# Autodesk Inventor assembly: sweeper
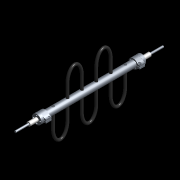
[picture p0: Inventor's stored thumbnail of the model, 180x180]
Saved by Autodesk Inventor 2015 SP1 (Build 190203100, 203)
## iProperties
Created: 2015-01-25
Part Number: sweeper
Document SubType Name: Assembly
Designer: rihoobler
Author: rihoobler
## Documents named in this file (7)
- C:\Users\datenney\Documents\GitHub\CAD\SerenityMk.2\sweeper.iam
- C:\Users\datenney\Documents\GitHub\CAD\SerenityMk.2\Sweeper tube.ipt
- C:\Users\datenney\Documents\GitHub\CAD\SerenityMk.2\Surgical.ipt
- C:\Users\datenney\Documents\GitHub\CAD\SerenityMk.2\Imported Components\tetrix_739077_2012\tetrix_739077_2012.ipt
- C:\Users\datenney\Documents\GitHub\CAD\SerenityMk.2\Imported Components\tetrix_739172_2012\tetrix_739172_2012.iam
- C:\Users\datenney\Documents\GitHub\CAD\SerenityMk.2\Imported Components\tetrix_739088_2012\tetrix_739088_2012.ipt
- C:\Users\datenney\Documents\GitHub\CAD\SerenityMk.2\Imported Components\tetrix_739101_2012\tetrix_739101_2012.ipt
## Components (16 placed, 6 different names)
1. Sweeper tube:1 — Mate:1, Mate:2, Mate:4, Mate:5, Mate:7, Mate:8, Mate:11, Mate:13, Mate:14, Insert:1, Insert:2
2. Surgical:1 — Mate:3, Mate:4, Mate:5, Mate:6
3. Surgical:2 — Mate:6, Mate:7, Mate:8, Mate:9, Mate:10
4. Surgical:3 — Mate:1, Mate:2, Flush:1, Mate:3, Flush:2
5. Surgical:4 — Mate:9, Mate:10, Mate:11, Mate:12
6. Surgical:5 — Mate:12, Mate:13, Mate:14
7. tetrix_739077_2012:1 — Insert:2, Insert:4
8. tetrix_739077_2012:2 — Insert:1, Flush:2, Insert:3
9. tetrix_739172_2012:1 [sub-assembly] — Insert:4, Mate:15, Flush:3, Insert:7
10. tetrix_739172_2012:2 [sub-assembly] — Insert:3, Mate:16, Flush:4, Insert:5
11. tetrix_739088_2012:1 — Mate:16, Flush:4
12. tetrix_739088_2012:2 — Mate:15, Flush:3
13. tetrix_739101_2012:1 — Insert:6
14. tetrix_739101_2012:2 — Insert:5, Insert:6
15. tetrix_739101_2012:3 — Insert:8
16. tetrix_739101_2012:4 — Insert:7, Insert:8
## Relationships (28: Mate 16, Insert 8, Flush 4)
- Mate:1: Sweeper tube:1 ↔ Surgical:3
- Mate:2: Sweeper tube:1 ↔ Surgical:3
- Flush:1: Surgical:3
- Mate:3: Surgical:1 ↔ Surgical:3
- Mate:4: Sweeper tube:1 ↔ Surgical:1
- Mate:5: Sweeper tube:1 ↔ Surgical:1
- Mate:6: Surgical:1 ↔ Surgical:2
- Mate:7: Sweeper tube:1 ↔ Surgical:2
- Mate:8: Sweeper tube:1 ↔ Surgical:2
- Mate:9: Surgical:2 ↔ Surgical:4
- Mate:10: Surgical:2 ↔ Surgical:4
- Mate:11: Sweeper tube:1 ↔ Surgical:4
- Mate:12: Surgical:4 ↔ Surgical:5
- Mate:13: Sweeper tube:1 ↔ Surgical:5
- Mate:14: Sweeper tube:1 ↔ Surgical:5
- Insert:1: Sweeper tube:1 ↔ tetrix_739077_2012:2
- Insert:2: Sweeper tube:1 ↔ tetrix_739077_2012:1
- Flush:2: Surgical:3 ↔ tetrix_739077_2012:2
- Insert:3: tetrix_739077_2012:2 ↔ tetrix_739172_2012:2
- Insert:4: tetrix_739077_2012:1 ↔ tetrix_739172_2012:1
- Mate:15: tetrix_739172_2012:1 ↔ tetrix_739088_2012:2
- Flush:3 (-50.8 mm): tetrix_739172_2012:1 ↔ tetrix_739088_2012:2
- Mate:16: tetrix_739172_2012:2 ↔ tetrix_739088_2012:1
- Flush:4 (-50.8 mm): tetrix_739172_2012:2 ↔ tetrix_739088_2012:1
- Insert:5: tetrix_739172_2012:2 ↔ tetrix_739101_2012:2
- Insert:6: tetrix_739101_2012:1 ↔ tetrix_739101_2012:2
- Insert:7: tetrix_739172_2012:1 ↔ tetrix_739101_2012:4
- Insert:8: tetrix_739101_2012:3 ↔ tetrix_739101_2012:4
